# Autodesk Inventor assembly: Internal Narrow Panels
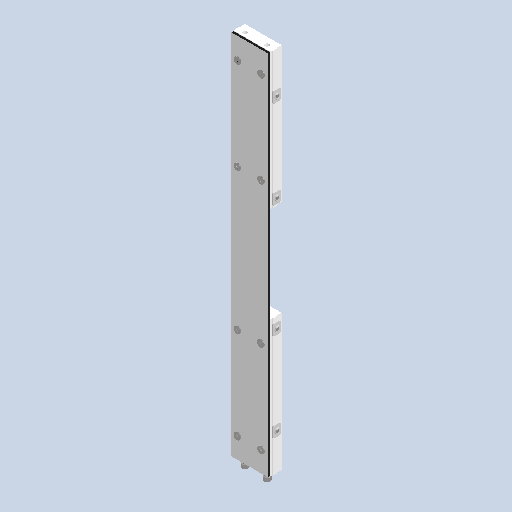
[picture p0: Inventor's stored thumbnail of the model, 512x512]
Saved by Autodesk Inventor 2024 (Build 280153000, 153)
## iProperties
Created: 2024-09-28
Part Number: Internal Narrow Panels
Document SubType Name: Assembly
Designer: Ishaan
Author: Ishaan
## Documents named in this file (8)
- E:\Projects\Axiom--IDEX-3D-Printer\CAD\08 - Side Panelling\Internal Narrow Panels.iam
- E:\Projects\Axiom--IDEX-3D-Printer\CAD\08 - Side Panelling\Internal narrow panel supports.ipt
- E:\Projects\Axiom--IDEX-3D-Printer\CAD\08 - Side Panelling\Narrow Internal Vertical Side Panels.ipt
- E:\Projects\Axiom--IDEX-3D-Printer\CAD\00 - COTS Components\Hardware\SHCSM5x12.ipt
- E:\Projects\Axiom--IDEX-3D-Printer\CAD\00 - COTS Components\Hardware\M5 LOCKNUT.ipt
- E:\Projects\Axiom--IDEX-3D-Printer\CAD\00 - COTS Components\Hardware\M5 T SLOT NUT.ipt
- E:\Projects\Axiom--IDEX-3D-Printer\CAD\00 - COTS Components\Hardware\Low Profile M5x16.ipt
- E:\Projects\Axiom--IDEX-3D-Printer\CAD\00 - COTS Components\Hardware\SHCSM5x16.ipt
## Components (41 placed, 7 different names)
1. Internal narrow panel supports:1 — Insert:1, Insert:2, Insert:3, Insert:4, Insert:13, Insert:14, Insert:15, Insert:16, Insert:17, Insert:18, Insert:19, Insert:20, Insert:27, Insert:28, Angle:1, Angle:2, Angle:9, Angle:10, Angle:11, Angle:12, Insert:29, Insert:30, Insert:35, Insert:36, Angle:13, Angle:14, Angle:15, Angle:19, Angle:20, Insert:47, Insert:48
2. Internal narrow panel supports:2 — Insert:5, Insert:6, Insert:7, Insert:8, Insert:9, Insert:10, Insert:11, Insert:12, Insert:21, Insert:22, Insert:23, Insert:24, Insert:25, Insert:26, Angle:3, Angle:4, Angle:5, Angle:6, Angle:7, Angle:8, Insert:31, Insert:32, Insert:33, Insert:34, Angle:16, Angle:17, Angle:18
3. Narrow Internal Vertical Side Panels:1 — Insert:1, Insert:2, Insert:3, Insert:4, Insert:5, Insert:6, Insert:7, Insert:8, Insert:37, Insert:38, Insert:39, Insert:40, Insert:41, Insert:42, Insert:43, Insert:44
4. SHCSM5x12:1 — Insert:12
5. SHCSM5x12:2 — Insert:11
6. SHCSM5x12:3 — Insert:10
7. SHCSM5x12:4 — Insert:9
8. SHCSM5x12:5 — Insert:13
9. SHCSM5x12:6 — Insert:14
10. SHCSM5x12:7 — Insert:15
11. SHCSM5x12:8 — Insert:16
12. M5 LOCKNUT:1 — Insert:19, Angle:9
13. M5 LOCKNUT:2 — Insert:23, Angle:6
14. M5 LOCKNUT:3 — Insert:24, Angle:5
15. M5 LOCKNUT:4 — Insert:28, Angle:2
16. M5 LOCKNUT:5 — Insert:26, Angle:3
17. M5 LOCKNUT:6 — Insert:22, Angle:7
18. M5 LOCKNUT:7 — Insert:18, Angle:12
19. M5 LOCKNUT:8 — Insert:20, Angle:10
20. M5 LOCKNUT:9 — Insert:21, Angle:8
21. M5 LOCKNUT:10 — Insert:27, Angle:1
22. M5 LOCKNUT:11 — Insert:25, Angle:4
23. M5 LOCKNUT:12 — Insert:17, Angle:11
24. M5 T SLOT NUT:1 — Insert:34, Angle:15
25. M5 T SLOT NUT:2 — Insert:36, Angle:13
26. M5 T SLOT NUT:3 — Insert:35, Angle:14
27. M5 T SLOT NUT:4 — Insert:30, Angle:20
28. M5 T SLOT NUT:5 — Insert:29, Angle:19
29. M5 T SLOT NUT:6 — Insert:31, Angle:18
30. M5 T SLOT NUT:7 — Insert:32, Angle:17
31. M5 T SLOT NUT:8 — Insert:33, Angle:16
32. Low Profile M5x16:1 — Insert:42
33. Low Profile M5x16:2 — Insert:41
34. Low Profile M5x16:3 — Insert:38
35. Low Profile M5x16:4 — Insert:37
36. Low Profile M5x16:5 — Insert:39
37. Low Profile M5x16:6 — Insert:40
38. Low Profile M5x16:7 — Insert:43
39. Low Profile M5x16:8 — Insert:44
40. SHCSM5x16:1 — Insert:48
41. SHCSM5x16:2 — Insert:47
## Relationships (66: Insert 46, Angle 20)
- Insert:1: Internal narrow panel supports:1 ↔ Narrow Internal Vertical Side Panels:1
- Insert:2: Internal narrow panel supports:1 ↔ Narrow Internal Vertical Side Panels:1
- Insert:3: Internal narrow panel supports:1 ↔ Narrow Internal Vertical Side Panels:1
- Insert:4: Internal narrow panel supports:1 ↔ Narrow Internal Vertical Side Panels:1
- Insert:5: Internal narrow panel supports:2 ↔ Narrow Internal Vertical Side Panels:1
- Insert:6: Internal narrow panel supports:2 ↔ Narrow Internal Vertical Side Panels:1
- Insert:7: Internal narrow panel supports:2 ↔ Narrow Internal Vertical Side Panels:1
- Insert:8: Internal narrow panel supports:2 ↔ Narrow Internal Vertical Side Panels:1
- Insert:9: Internal narrow panel supports:2 ↔ SHCSM5x12:4
- Insert:10: Internal narrow panel supports:2 ↔ SHCSM5x12:3
- Insert:11: Internal narrow panel supports:2 ↔ SHCSM5x12:2
- Insert:12: Internal narrow panel supports:2 ↔ SHCSM5x12:1
- Insert:13: Internal narrow panel supports:1 ↔ SHCSM5x12:5
- Insert:14: Internal narrow panel supports:1 ↔ SHCSM5x12:6
- Insert:15: Internal narrow panel supports:1 ↔ SHCSM5x12:7
- Insert:16: Internal narrow panel supports:1 ↔ SHCSM5x12:8
- Insert:17: Internal narrow panel supports:1 ↔ M5 LOCKNUT:12
- Insert:18: Internal narrow panel supports:1 ↔ M5 LOCKNUT:7
- Insert:19: Internal narrow panel supports:1 ↔ M5 LOCKNUT:1
- Insert:20: Internal narrow panel supports:1 ↔ M5 LOCKNUT:8
- Insert:21: Internal narrow panel supports:2 ↔ M5 LOCKNUT:9
- Insert:22: Internal narrow panel supports:2 ↔ M5 LOCKNUT:6
- Insert:23: Internal narrow panel supports:2 ↔ M5 LOCKNUT:2
- Insert:24: Internal narrow panel supports:2 ↔ M5 LOCKNUT:3
- Insert:25: Internal narrow panel supports:2 ↔ M5 LOCKNUT:11
- Insert:26: Internal narrow panel supports:2 ↔ M5 LOCKNUT:5
- Insert:27: Internal narrow panel supports:1 ↔ M5 LOCKNUT:10
- Insert:28: Internal narrow panel supports:1 ↔ M5 LOCKNUT:4
- Angle:1 (0 deg): Internal narrow panel supports:1 ↔ M5 LOCKNUT:10
- Angle:2 (0 deg): Internal narrow panel supports:1 ↔ M5 LOCKNUT:4
- Angle:3 (0 deg): Internal narrow panel supports:2 ↔ M5 LOCKNUT:5
- Angle:4 (0 deg): Internal narrow panel supports:2 ↔ M5 LOCKNUT:11
- Angle:5 (0 deg): Internal narrow panel supports:2 ↔ M5 LOCKNUT:3
- Angle:6 (0 deg): Internal narrow panel supports:2 ↔ M5 LOCKNUT:2
- Angle:7 (0 deg): Internal narrow panel supports:2 ↔ M5 LOCKNUT:6
- Angle:8 (0 deg): Internal narrow panel supports:2 ↔ M5 LOCKNUT:9
- Angle:9 (0 deg): Internal narrow panel supports:1 ↔ M5 LOCKNUT:1
- Angle:10 (0 deg): Internal narrow panel supports:1 ↔ M5 LOCKNUT:8
- Angle:11 (0 deg): Internal narrow panel supports:1 ↔ M5 LOCKNUT:12
- Angle:12 (0 deg): Internal narrow panel supports:1 ↔ M5 LOCKNUT:7
- Insert:29 (2 mm): Internal narrow panel supports:1 ↔ M5 T SLOT NUT:5
- Insert:30 (2 mm): Internal narrow panel supports:1 ↔ M5 T SLOT NUT:4
- Insert:31 (2 mm): Internal narrow panel supports:2 ↔ M5 T SLOT NUT:6
- Insert:32 (2 mm): Internal narrow panel supports:2 ↔ M5 T SLOT NUT:7
- Insert:33 (2 mm): Internal narrow panel supports:2 ↔ M5 T SLOT NUT:8
- Insert:34 (2 mm): Internal narrow panel supports:2 ↔ M5 T SLOT NUT:1
- Insert:35 (2 mm): Internal narrow panel supports:1 ↔ M5 T SLOT NUT:3
- Insert:36 (2 mm): Internal narrow panel supports:1 ↔ M5 T SLOT NUT:2
- Angle:13 (0 deg): Internal narrow panel supports:1 ↔ M5 T SLOT NUT:2
- Angle:14 (0 deg): Internal narrow panel supports:1 ↔ M5 T SLOT NUT:3
- Angle:15 (0 deg): Internal narrow panel supports:1 ↔ M5 T SLOT NUT:1
- Angle:16 (0 deg): Internal narrow panel supports:2 ↔ M5 T SLOT NUT:8
- Angle:17 (0 deg): Internal narrow panel supports:2 ↔ M5 T SLOT NUT:7
- Angle:18 (0 deg): Internal narrow panel supports:2 ↔ M5 T SLOT NUT:6
- Angle:19 (0 deg): Internal narrow panel supports:1 ↔ M5 T SLOT NUT:5
- Angle:20 (0 deg): Internal narrow panel supports:1 ↔ M5 T SLOT NUT:4
- Insert:37: Narrow Internal Vertical Side Panels:1 ↔ Low Profile M5x16:4
- Insert:38: Narrow Internal Vertical Side Panels:1 ↔ Low Profile M5x16:3
- Insert:39: Narrow Internal Vertical Side Panels:1 ↔ Low Profile M5x16:5
- Insert:40: Narrow Internal Vertical Side Panels:1 ↔ Low Profile M5x16:6
- Insert:41: Narrow Internal Vertical Side Panels:1 ↔ Low Profile M5x16:2
- Insert:42: Narrow Internal Vertical Side Panels:1 ↔ Low Profile M5x16:1
- Insert:43: Narrow Internal Vertical Side Panels:1 ↔ Low Profile M5x16:7
- Insert:44: Narrow Internal Vertical Side Panels:1 ↔ Low Profile M5x16:8
- Insert:47 (6.35 mm): Internal narrow panel supports:1 ↔ SHCSM5x16:2
- Insert:48 (6.35 mm): Internal narrow panel supports:1 ↔ SHCSM5x16:1
